# Autodesk Inventor assembly: Turret
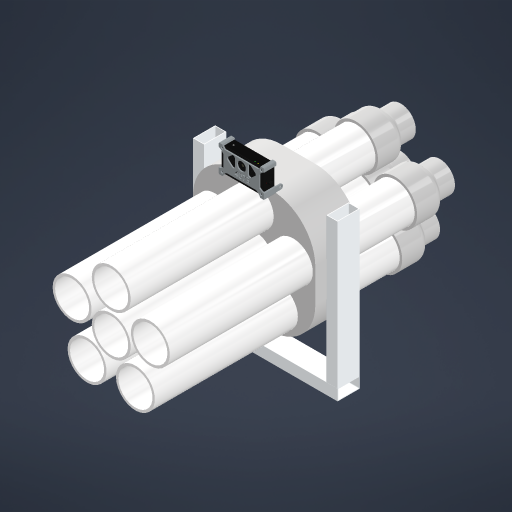
[picture p0: Inventor's stored thumbnail of the model, 512x512]
Saved by Autodesk Inventor 2023 (Build 270158000, 158)
## iProperties
Created: 2022-06-21
Part Number: Turret
Document SubType Name: Assembly
Designer: timmy
Author: timmy
## Documents named in this file (5)
- R:\Inventor\RoboCatz\T-Shirt\Rev2-Better\Turret.iam
- R:\Inventor\RoboCatz\T-Shirt\Rev2-Better\ShooterMount.ipt
- R:\Inventor\RoboCatz\T-Shirt\Rev2-Better\Limelight.iam
- R:\Inventor\RoboCatz\T-Shirt\Rev2-Better\am-3214 2x1x0625 wall tubing.ipt
- R:\Inventor\RoboCatz\T-Shirt\Rev2-Better\Shooter-pipes.iam
## Components (11 placed, 4 different names)
1. ShooterMount:1 — Mate:7, Flush:6, Mate:8, Mate:10, Mate:11, Mate:12, Angle:1, Mate:13, Mate:14, Mate:15, Mate:16, Mate:17, Mate:18
2. Limelight:1 [sub-assembly] — Mate:7, Flush:6
3. am-3214 2x1x0625 wall tubing:1 — Mate:10, Flush:7, Mate:12, Flush:8
4. am-3214 2x1x0625 wall tubing:2 — Mate:8, Mate:9, Flush:7, Mate:11, Flush:9, Angle:1
5. am-3214 2x1x0625 wall tubing:3 — Mate:9, Flush:8, Flush:9
6. Shooter-pipes:1 [sub-assembly] — Mate:15, Flush:10
7. Shooter-pipes:2 [sub-assembly] — Mate:14, Flush:11
8. Shooter-pipes:3 [sub-assembly] — Mate:16, Flush:14
9. Shooter-pipes:4 [sub-assembly] — Mate:17, Flush:13
10. Shooter-pipes:5 [sub-assembly] — Mate:13, Flush:10, Flush:11, Flush:12, Flush:13, Flush:14
11. Shooter-pipes:6 [sub-assembly] — Mate:18, Flush:12
## Relationships (22: Mate 12, Flush 9, Angle 1)
- Mate:7: ShooterMount:1 ↔ Limelight:1
- Flush:6: ShooterMount:1 ↔ Limelight:1
- Mate:8: ShooterMount:1 ↔ am-3214 2x1x0625 wall tubing:2
- Mate:9: am-3214 2x1x0625 wall tubing:2 ↔ am-3214 2x1x0625 wall tubing:3
- Mate:10: ShooterMount:1 ↔ am-3214 2x1x0625 wall tubing:1
- Flush:7: am-3214 2x1x0625 wall tubing:1 ↔ am-3214 2x1x0625 wall tubing:2
- Mate:11: ShooterMount:1 ↔ am-3214 2x1x0625 wall tubing:2
- Mate:12: ShooterMount:1 ↔ am-3214 2x1x0625 wall tubing:1
- Flush:8: am-3214 2x1x0625 wall tubing:1 ↔ am-3214 2x1x0625 wall tubing:3
- Flush:9: am-3214 2x1x0625 wall tubing:2 ↔ am-3214 2x1x0625 wall tubing:3
- Angle:1 (0 deg): ShooterMount:1 ↔ am-3214 2x1x0625 wall tubing:2
- Mate:13: ShooterMount:1 ↔ Shooter-pipes:5
- Mate:14: ShooterMount:1 ↔ Shooter-pipes:2
- Mate:15: ShooterMount:1 ↔ Shooter-pipes:1
- Mate:16: ShooterMount:1 ↔ Shooter-pipes:3
- Mate:17: ShooterMount:1 ↔ Shooter-pipes:4
- Mate:18: ShooterMount:1 ↔ Shooter-pipes:6
- Flush:10: Shooter-pipes:1 ↔ Shooter-pipes:5
- Flush:11: Shooter-pipes:2 ↔ Shooter-pipes:5
- Flush:12: Shooter-pipes:5 ↔ Shooter-pipes:6
- Flush:13: Shooter-pipes:4 ↔ Shooter-pipes:5
- Flush:14: Shooter-pipes:3 ↔ Shooter-pipes:5
